# Autodesk Inventor assembly: Assem_Soln
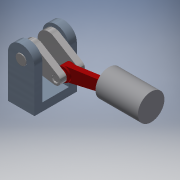
[picture p0: Inventor's stored thumbnail of the model, 180x180]
Saved by Autodesk Inventor 2016 (Build 200138000, 138)
## iProperties
Created: 2017-07-15
Part Number: Assem_Soln
Document SubType Name: Assembly
Designer: bobbyl
Author: bobbyl
## Documents named in this file (6)
- C:\Users\bobbyl\Desktop\CAD QuickStart 2017\Lesson 2\Piston_Example\Assem_Soln.iam
- C:\Users\bobbyl\Desktop\CAD QuickStart 2017\Lesson 2\Piston_Example\Base_Block.ipt
- C:\Users\bobbyl\Desktop\CAD QuickStart 2017\Lesson 2\Piston_Example\Crank.ipt
- C:\Users\bobbyl\Desktop\CAD QuickStart 2017\Lesson 2\Piston_Example\Connector_Rod.ipt
- C:\Users\bobbyl\Desktop\CAD QuickStart 2017\Lesson 2\Piston_Example\Piston.ipt
- C:\Users\bobbyl\Desktop\CAD QuickStart 2017\Lesson 2\Piston_Example\Cylinder.ipt
## Components (5 placed, 5 different names)
1. Base_Block:1 — Rotational:1, Flush:1, Flush:2
2. Crank:1 — Rotational:1, Rotational:2
3. Connector_Rod:1 — Rotational:2, Rotational:3
4. Piston:1 — Rotational:3, Mate:1
5. Cylinder:1 — Mate:1, Flush:1, Flush:2
## Relationships (6: RevoluteJoint 3, Flush 2, Mate 1)
- Rotational:1 [RevoluteJoint]: Base_Block:1 ↔ Crank:1
- Rotational:2 [RevoluteJoint]: Crank:1 ↔ Connector_Rod:1
- Rotational:3 [RevoluteJoint]: Connector_Rod:1 ↔ Piston:1
- Mate:1: Piston:1 ↔ Cylinder:1
- Flush:1 (180 mm): Base_Block:1 ↔ Cylinder:1
- Flush:2 (85 mm): Base_Block:1 ↔ Cylinder:1
